# Autodesk Inventor assembly: 5 Barras Version 0
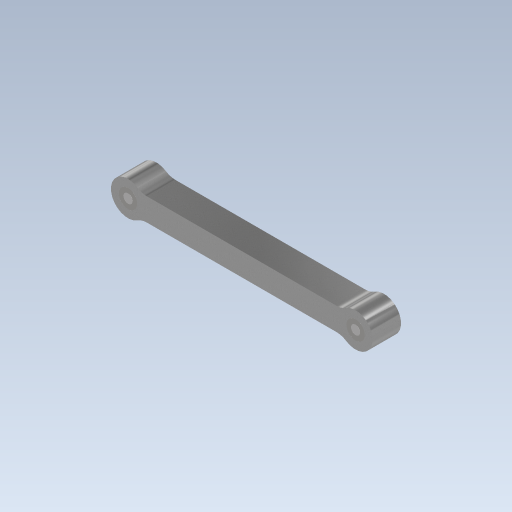
[picture p0: Inventor's stored thumbnail of the model, 512x512]
Saved by Autodesk Inventor 2024.2 (Build 282272000, 272)
## iProperties
Created: 2025-02-06
Part Number: 5 Barras Version 0
Document SubType Name: Assembly
Designer: jp.reyesf
Author: jp.reyesf
## Documents named in this file (5)
- C:\Users\jp.reyesf\Desktop\Master-Thesis\five_bar\assets\CAD\Robot\Subassemblies\Distal Link 2.iam
- C:\Users\jp.reyesf\Desktop\Master-Thesis\five_bar\assets\CAD\Robot\Distal Link 1.ipt
- C:\Users\jp.reyesf\Desktop\Master-Thesis\five_bar\assets\CAD\Robot\Spacer.ipt
- C:\Users\jp.reyesf\Desktop\Master-Thesis\five_bar\assets\CAD\Robot\Bearing.ipt
- C:\Users\jp.reyesf\Desktop\Master-Thesis\five_bar\assets\CAD\Robot\Subassemblies\DummyBar.ipt
## Components (9 placed, 4 different names)
1. Distal Link 1:1 — Mate:31, Mate:32, Flush:2, Flush:3, Mate:33, Angle:1, Flush:4, Mate:34, Mate:35, Flush:5, Flush:6
2. Spacer:5 — Mate:32
3. Bearing:10 — Flush:2
4. Bearing:11
5. Spacer:6 — Mate:31
6. Bearing:12 — Flush:3
7. Bearing:13
8. DummyBar:1 — Mate:34, Flush:5
9. DummyBar:2 — Mate:35, Flush:6
## Relationships (19: Mate 13, Flush 5, Angle 1)
- [Mate]: Spacer:5 ↔ Bearing:10
- [Mate]: Spacer:5 ↔ Bearing:11
- [Mate]: Spacer:5 ↔ Bearing:10
- [Mate]: Spacer:5 ↔ Bearing:11
- [Mate]: Spacer:6 ↔ Bearing:12
- [Mate]: Spacer:6 ↔ Bearing:13
- [Mate]: Spacer:6 ↔ Bearing:12
- [Mate]: Spacer:6 ↔ Bearing:13
- Mate:31: Distal Link 1:1 ↔ Spacer:6
- Mate:32: Distal Link 1:1 ↔ Spacer:5
- Flush:2: Distal Link 1:1 ↔ Bearing:10
- Flush:3: Distal Link 1:1 ↔ Bearing:12
- Mate:33: Distal Link 1:1
- Angle:1 (180 deg): Distal Link 1:1
- Flush:4: Distal Link 1:1
- Mate:34: Distal Link 1:1 ↔ DummyBar:1
- Mate:35: Distal Link 1:1 ↔ DummyBar:2
- Flush:5: Distal Link 1:1 ↔ DummyBar:1
- Flush:6: Distal Link 1:1 ↔ DummyBar:2
## Named parameters: d30_d14 = 0 mm, d31_d15 = 0 mm, d32_d16 = 0 mm, d33_d17 = 0 mm, d34_d14 = 0 mm, d35_d15 = 0 mm, d36_d16 = 0 mm, d37_d17 = 0 mm
